# Autodesk Inventor assembly: AM14U4 Square Frame Half
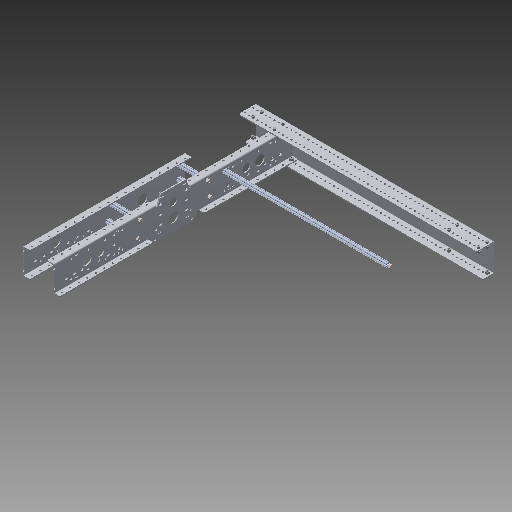
[picture p0: Inventor's stored thumbnail of the model, 512x512]
Saved by Autodesk Inventor 2017 (Build 210142000, 142)
## iProperties
Part Number: AM14U4 Square Frame Half
Material: 一般
Document SubType Name: Assembly
Designer: IJA
Author: IJA
Revision Number: ANY
## Documents named in this file (9)
- D:\Works\Robot2\AM14U4 Square Frame Half.iam
- D:\Works\Robot2\am-xxxx AM14U4 End Plate Square.ipt
- D:\Works\Robot2\am-xxxx AM14U4 Inside Plate Square.ipt
- D:\Works\Robot2\am-1002 and am-1042 10-32 x 0500 and Nylock Nut Assembly.iam
- D:\Works\Robot2\FHTS 0.25-20-0.75_FHTS 0.25-20-G-0.75-C.ipt
- D:\Works\Robot2\3.375in Churro.ipt
- D:\Works\Robot2\19.25in Churro.ipt
- D:\Works\Robot2\am-xxxx AM14U4 Outside Plate Square_DefaultSM-FLAT-PATTERN_MIR2.ipt
- D:\Works\Robot2\am-xxxx AM14U4 Inside Plate Square2.ipt
## Components (31 placed, 31 different names)
1. am-xxxx AM14U4 End Plate Square_82 — 貼合:2, 貼合:3
2. am-xxxx AM14U4 Inside Plate Square_84
3. am-1002 and am-1042 10-32 x 0500 and Nylock Nut Assembly_85 [sub-assembly] — 貼合:2
4. am-1002 and am-1042 10-32 x 0500 and Nylock Nut Assembly_86 [sub-assembly] — 貼合:3
5. am-1002 and am-1042 10-32 x 0500 and Nylock Nut Assembly_87 [sub-assembly]
6. am-1002 and am-1042 10-32 x 0500 and Nylock Nut Assembly_88 [sub-assembly]
7. am-1002 and am-1042 10-32 x 0500 and Nylock Nut Assembly_89 [sub-assembly]
8. am-1002 and am-1042 10-32 x 0500 and Nylock Nut Assembly_90 [sub-assembly]
9. am-1002 and am-1042 10-32 x 0500 and Nylock Nut Assembly_91 [sub-assembly]
10. am-1002 and am-1042 10-32 x 0500 and Nylock Nut Assembly_92 [sub-assembly]
11. am-1002 and am-1042 10-32 x 0500 and Nylock Nut Assembly_93 [sub-assembly]
12. FHTS 0.25-20-0.75_FHTS 0.25-20-G-0.75-C_94
13. FHTS 0.25-20-0.75_FHTS 0.25-20-G-0.75-C_95
14. FHTS 0.25-20-0.75_FHTS 0.25-20-G-0.75-C_96
15. FHTS 0.25-20-0.75_FHTS 0.25-20-G-0.75-C_97
16. FHTS 0.25-20-0.75_FHTS 0.25-20-G-0.75-C_98
17. FHTS 0.25-20-0.75_FHTS 0.25-20-G-0.75-C_99
18. FHTS 0.25-20-0.75_FHTS 0.25-20-G-0.75-C_100
19. FHTS 0.25-20-0.75_FHTS 0.25-20-G-0.75-C_101
20. 3.375in Churro_102
21. 3.375in Churro_103
22. 3.375in Churro_104
23. 3.375in Churro_105
24. am-1002 and am-1042 10-32 x 0500 and Nylock Nut Assembly_106 [sub-assembly]
25. am-1002 and am-1042 10-32 x 0500 and Nylock Nut Assembly_107 [sub-assembly]
26. am-1002 and am-1042 10-32 x 0500 and Nylock Nut Assembly_108 [sub-assembly]
27. 19.25in Churro_109
28. FHTS 0.25-20-0.75_FHTS 0.25-20-G-0.75-C_110
29. FHTS 0.25-20-0.75_FHTS 0.25-20-G-0.75-C_111
30. am-xxxx AM14U4 Outside Plate Square_DefaultSM-FLAT-PATTERN_MIR2:1
31. am-xxxx AM14U4 Inside Plate Square2:1
## Relationships (3: Mate 2, Angle 1)
- 貼合:2 [Mate]: am-xxxx AM14U4 End Plate Square_82 ↔ am-1002 and am-1042 10-32 x 0500 and Nylock Nut Assembly_85
- 貼合:3 [Mate]: am-xxxx AM14U4 End Plate Square_82 ↔ am-1002 and am-1042 10-32 x 0500 and Nylock Nut Assembly_86
- [Angle] (0 deg): am-xxxx AM14U4 Inside Plate Square_84 ↔ am-xxxx AM14U4 Outside Plate Square_DefaultSM-FLAT-PATTERN_MIR2:1
## Named parameters: d3_d2 = 0 deg
